# Autodesk Inventor assembly: ASY ДМФ 040 кольцо под шпильки КОРМА
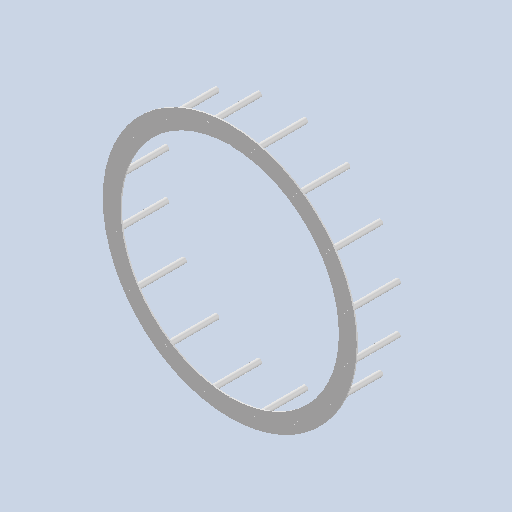
[picture p0: Inventor's stored thumbnail of the model, 512x512]
Saved by Autodesk Inventor 2025 (Build 290162010, 162A)
## iProperties
Created: 2024-05-08
Part Number: ASY ДМФ 040 кольцо под шпильки КОРМА
Document SubType Name: Assembly
Designer: pokla
Stock Number: ДМФ 040 кольцо под шпильки КОРМА
Author: pokla
## Documents named in this file (4)
- C:\Users\pokla\Documents\Inventor\ДФО\ДМФ\DMF-Disk-Micro-Filter\DMF old version\ASY ДМФ 070 кольцо под шпильки КОРМА наружное.iam
- C:\Users\pokla\Documents\Inventor\ДФО\ДМФ\DMF-Disk-Micro-Filter\DMF old version\ДМФ 041 кольцо под шпильки КОРМА.ipt
- C:\Users\pokla\Documents\Inventor\ДФО\ДМФ\DMF-Disk-Micro-Filter\DMF old version\ДМФ 042 шпилька 1.ipt
- C:\Users\pokla\Documents\Inventor\ДФО\ДМФ\DMF-Disk-Micro-Filter\DMF old version\ДМФ 000 размеры.ipt
## Components (17 placed, 2 different names)
1. ДМФ 041 кольцо под шпильки КОРМА.ipt:1 — Rigid:1
2. ДМФ 042 шпилька 1.ipt:1 — Rigid:1
3. ДМФ 042 шпилька 1.ipt:2
4. ДМФ 042 шпилька 1.ipt:3
5. ДМФ 042 шпилька 1.ipt:4
6. ДМФ 042 шпилька 1.ipt:5
7. ДМФ 042 шпилька 1.ipt:6
8. ДМФ 042 шпилька 1.ipt:7
9. ДМФ 042 шпилька 1.ipt:8
10. ДМФ 042 шпилька 1.ipt:9
11. ДМФ 042 шпилька 1.ipt:10
12. ДМФ 042 шпилька 1.ipt:11
13. ДМФ 042 шпилька 1.ipt:12
14. ДМФ 042 шпилька 1.ipt:13
15. ДМФ 042 шпилька 1.ipt:14
16. ДМФ 042 шпилька 1.ipt:15
17. ДМФ 042 шпилька 1.ipt:16
## Component patterns: (16 elements, first: ДМФ 042 шпилька 1.ipt:1)
## Relationships (1: WeldJoint 1)
- Rigid:1 [WeldJoint]: ДМФ 041 кольцо под шпильки КОРМА.ipt:1 ↔ ДМФ 042 шпилька 1.ipt:1
